# Autodesk Inventor assembly: POM_T5_08
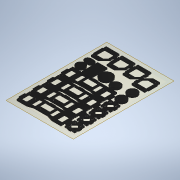
[picture p0: Inventor's stored thumbnail of the model, 180x180]
Saved by Autodesk Inventor 2020 (Build 240168000, 168)
## iProperties
Created: 2021-08-27
Part Number: POM_T5_08
Document SubType Name: Assembly
Designer: Masato
Author: Masato
## Documents named in this file (11)
- C:\Inventor\SUSTAINA-OP_0422\Cam\POM_T5_08.iam
- C:\Inventor\SUSTAINA-OP_0422\Cam\DisposableBoard.ipt
- C:\Inventor\SUSTAINA-OP_0422\UpperBody\Arm\UpperArm_diagonal.ipt
- C:\Inventor\SUSTAINA-OP_0422\SandBlastingJig\Trunk_servo_bottom_frame_SandBlastingJig.ipt
- C:\Inventor\SUSTAINA-OP_0422\SandBlastingJig\Leg_joint_slider_frame_SandBlastingJig_slider_front.ipt
- C:\Inventor\SUSTAINA-OP_0422\SandBlastingJig\Leg_joint_yaw_frame_SandBlastingJig.ipt
- C:\Inventor\SUSTAINA-OP_0422\SandBlastingJig\Outer_support_stand_SandBlastingJig.ipt
- C:\Inventor\SUSTAINA-OP_0422\SandBlastingJig\Shoulder_horn_frame_SandBlastingJig.ipt
- C:\Inventor\SUSTAINA-OP_0422\SandBlastingJig\Trunk_neck_frame_AND_Trunk_shoulder_frame_SandBlastingJig.ipt
- C:\Inventor\SUSTAINA-OP_0422\UpperBody\Arm\ForeArm_diagonal.ipt
- C:\Inventor\SUSTAINA-OP_0422\UpperBody\Trunk\Trunk_chest_frame.ipt
## Components (20 placed, 10 different names)
1. DisposableBoard:1 — メイト:2, メイト:1, フラッシュ:1, フラッシュ:2, メイト:7, メイト:8, メイト:9, メイト:30, メイト:31, メイト:32, メイト:33, メイト:34, メイト:35, 角度:6, 角度:8, 角度:9, 角度:10, メイト:36, フラッシュ:5, フラッシュ:6, メイト:37, フラッシュ:7, フラッシュ:8, 角度:11, 正接:3, 正接:6, メイト:39
2. Trunk_servo_bottom_frame_SandBlastingJig:1 — メイト:30, メイト:38, 正接:7, 正接:8
3. Leg_joint_slider_frame_SandBlastingJig_slider_front:1 — メイト:32, 角度:11, 正接:5, 正接:6, 正接:7
4. Leg_joint_yaw_frame_SandBlastingJig:1 — メイト:33, 角度:10, 正接:3, 正接:4, 正接:5
5. Outer_support_stand_SandBlastingJig:1 — メイト:35, 角度:9, 正接:8, 正接:9, 正接:10
6. Trunk_neck_frame_AND_Trunk_shoulder_frame_SandBlastingJig:1 — メイト:31, 角度:6, 正接:10, 正接:11
7. ForeArm_diagonal:4 — フラッシュ:9, メイト:39, メイト:40
8. UpperArm_diagonal:1 — メイト:7, メイト:8, メイト:9
9. UpperArm_diagonal:2
10. UpperArm_diagonal:3
11. UpperArm_diagonal:4 — 正接:1, フラッシュ:9
12. ForeArm_diagonal:1 — メイト:36, フラッシュ:5, フラッシュ:6
13. ForeArm_diagonal:2
14. ForeArm_diagonal:3 — メイト:40
15. Trunk_chest_frame:1 — メイト:37, フラッシュ:7, フラッシュ:8
16. Trunk_chest_frame:2
17. Trunk_chest_frame:3
18. Trunk_chest_frame:4 — 正接:2, 正接:4, メイト:38, 正接:9, 正接:11
19. Shoulder_horn_frame_SandBlastingJig:1 — メイト:34, 角度:8, 正接:1, 正接:2
20. Shoulder_horn_frame_SandBlastingJig:2
## Component patterns: (4 elements, first: UpperArm_diagonal:1), (3 elements, first: ForeArm_diagonal:1), (4 elements, first: Trunk_chest_frame:1), (2 elements, first: Shoulder_horn_frame_SandBlastingJig:1)
## Relationships (39: Mate 16, Tangent 11, Flush 7, Angle 5)
- メイト:2 [Mate]: DisposableBoard:1
- メイト:1 [Mate]: DisposableBoard:1
- フラッシュ:1 [Flush]: DisposableBoard:1
- フラッシュ:2 [Flush]: DisposableBoard:1
- メイト:7 [Mate]: DisposableBoard:1 ↔ UpperArm_diagonal:1
- メイト:8 [Mate] (2 mm): DisposableBoard:1 ↔ UpperArm_diagonal:1
- メイト:9 [Mate] (2 mm): DisposableBoard:1 ↔ UpperArm_diagonal:1
- メイト:30 [Mate]: DisposableBoard:1 ↔ Trunk_servo_bottom_frame_SandBlastingJig:1
- メイト:31 [Mate]: DisposableBoard:1 ↔ Trunk_neck_frame_AND_Trunk_shoulder_frame_SandBlastingJig:1
- メイト:32 [Mate]: DisposableBoard:1 ↔ Leg_joint_slider_frame_SandBlastingJig_slider_front:1
- メイト:33 [Mate]: DisposableBoard:1 ↔ Leg_joint_yaw_frame_SandBlastingJig:1
- メイト:34 [Mate]: DisposableBoard:1 ↔ Shoulder_horn_frame_SandBlastingJig:1
- メイト:35 [Mate]: DisposableBoard:1 ↔ Outer_support_stand_SandBlastingJig:1
- 角度:6 [Angle] (0 deg): DisposableBoard:1 ↔ Trunk_neck_frame_AND_Trunk_shoulder_frame_SandBlastingJig:1
- 角度:8 [Angle] (0 deg): DisposableBoard:1 ↔ Shoulder_horn_frame_SandBlastingJig:1
- 角度:9 [Angle] (0 deg): DisposableBoard:1 ↔ Outer_support_stand_SandBlastingJig:1
- 角度:10 [Angle] (0 deg): DisposableBoard:1 ↔ Leg_joint_yaw_frame_SandBlastingJig:1
- メイト:36 [Mate]: DisposableBoard:1 ↔ ForeArm_diagonal:1
- フラッシュ:5 [Flush] (2.5 mm): DisposableBoard:1 ↔ ForeArm_diagonal:1
- フラッシュ:6 [Flush] (3.5 mm): DisposableBoard:1 ↔ ForeArm_diagonal:1
- メイト:37 [Mate]: DisposableBoard:1 ↔ Trunk_chest_frame:1
- フラッシュ:7 [Flush] (2.5 mm): DisposableBoard:1 ↔ Trunk_chest_frame:1
- フラッシュ:8 [Flush] (1.5 mm): DisposableBoard:1 ↔ Trunk_chest_frame:1
- 正接:1 [Tangent] (2.5 mm): UpperArm_diagonal:4 ↔ Shoulder_horn_frame_SandBlastingJig:1
- 正接:2 [Tangent] (2.5 mm): Trunk_chest_frame:4 ↔ Shoulder_horn_frame_SandBlastingJig:1
- 角度:11 [Angle] (90 deg): DisposableBoard:1 ↔ Leg_joint_slider_frame_SandBlastingJig_slider_front:1
- 正接:3 [Tangent] (2.5 mm): DisposableBoard:1 ↔ Leg_joint_yaw_frame_SandBlastingJig:1
- 正接:4 [Tangent] (2.5 mm): Leg_joint_yaw_frame_SandBlastingJig:1 ↔ Trunk_chest_frame:4
- 正接:5 [Tangent] (2.5 mm): Leg_joint_slider_frame_SandBlastingJig_slider_front:1 ↔ Leg_joint_yaw_frame_SandBlastingJig:1
- 正接:6 [Tangent] (2.5 mm): DisposableBoard:1 ↔ Leg_joint_slider_frame_SandBlastingJig_slider_front:1
- メイト:38 [Mate] (2.5 mm): Trunk_servo_bottom_frame_SandBlastingJig:1 ↔ Trunk_chest_frame:4
- 正接:7 [Tangent] (2.5 mm): Trunk_servo_bottom_frame_SandBlastingJig:1 ↔ Leg_joint_slider_frame_SandBlastingJig_slider_front:1
- 正接:8 [Tangent] (2.5 mm): Trunk_servo_bottom_frame_SandBlastingJig:1 ↔ Outer_support_stand_SandBlastingJig:1
- 正接:9 [Tangent] (2.5 mm): Outer_support_stand_SandBlastingJig:1 ↔ Trunk_chest_frame:4
- 正接:10 [Tangent] (2.5 mm): Outer_support_stand_SandBlastingJig:1 ↔ Trunk_neck_frame_AND_Trunk_shoulder_frame_SandBlastingJig:1
- 正接:11 [Tangent] (2.5 mm): Trunk_neck_frame_AND_Trunk_shoulder_frame_SandBlastingJig:1 ↔ Trunk_chest_frame:4
- フラッシュ:9 [Flush]: ForeArm_diagonal:4 ↔ UpperArm_diagonal:4
- メイト:39 [Mate]: DisposableBoard:1 ↔ ForeArm_diagonal:4
- メイト:40 [Mate] (2.5 mm): ForeArm_diagonal:4 ↔ ForeArm_diagonal:3
